# Autodesk Inventor assembly: UR5withBarrett
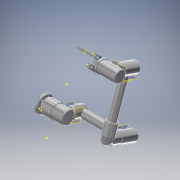
[picture p0: Inventor's stored thumbnail of the model, 180x180]
Saved by Autodesk Inventor 2016 (Build 200138000, 138)
## iProperties
Created: 2017-12-24
Part Number: UR5withBarrett
Document SubType Name: Assembly
Designer: kornbot
Author: kornbot
## Documents named in this file (15)
- C:\Users\kornbot\Documents\UR5withBarrett.iam
- C:\Users\kornbot\Documents\UR5 Joint base connection.ipt
- C:\Users\kornbot\Documents\UR5 base2.ipt
- C:\Users\kornbot\Documents\UR5 upper joint shoulder.ipt
- C:\Users\kornbot\Documents\UR5 joint shoulder 2.ipt
- C:\Users\kornbot\Documents\UR5 extended arm.ipt
- C:\Users\kornbot\Documents\UR5 joint elbow2.ipt
- C:\Users\kornbot\Documents\UR5 joint elbow3.ipt
- C:\Users\kornbot\Documents\UR5 Joint to wrist.ipt
- C:\Users\kornbot\Documents\UR5 End to wrist.ipt
- C:\Users\kornbot\Documents\UR5 Wrist Rotation.ipt
- C:\Users\kornbot\Documents\UR5 Palm.ipt
- C:\Users\kornbot\Documents\UR5 finger.ipt
- C:\Users\kornbot\Documents\UR5  finger lead.ipt
- C:\Users\kornbot\Documents\UR5 End finger.ipt
## Components (23 placed, 14 different names)
1. UR5 base2:1 — Rotational:1
2. UR5 Joint base connection:1 — Rotational:1, Rigid:1, Rigid:2
3. UR5 Joint base connection:2 — Rigid:1
4. UR5 upper joint shoulder:1 — Rigid:2, Rotational:2
5. UR5 joint shoulder 2:1 — Rotational:2, Rigid:3
6. UR5 joint shoulder 2:2 — Rigid:3, Rotational:3
7. UR5 extended arm:1 — Rotational:3, Rigid:4
8. UR5 joint elbow3:1 — Rigid:4, Rotational:4
9. UR5 Joint to wrist:1 — Rotational:4, Rigid:5
10. UR5 End to wrist:1 — Rigid:5, Rigid:6
11. UR5 joint elbow2:1 — Rigid:6, Rotational:5
12. UR5 joint elbow2:2 — Rotational:5, Rotational:6
13. UR5 Wrist Rotation:1 — Rotational:6, Rotational:7
14. UR5 Palm:1 — Rotational:7, Rotational:8, Rotational:9, Rigid:7
15. UR5 finger:1 — Rotational:9, Rotational:12
16. UR5 finger:2 — Rigid:7, Rotational:10
17. UR5 finger:3 — Rotational:8, Rotational:11
18. UR5  finger lead:1 — Rotational:10, Rotational:13
19. UR5  finger lead:2 — Rotational:12, Rotational:15
20. UR5  finger lead:3 — Rotational:11, Rotational:14
21. UR5 End finger:1 — Rotational:13
22. UR5 End finger:2 — Rotational:14
23. UR5 End finger:3 — Rotational:15
## Relationships (22: RevoluteJoint 15, WeldJoint 7)
- Rotational:1 [RevoluteJoint]: UR5 base2:1 ↔ UR5 Joint base connection:1
- Rigid:1 [WeldJoint]: UR5 Joint base connection:1 ↔ UR5 Joint base connection:2
- Rigid:2 [WeldJoint]: UR5 Joint base connection:1 ↔ UR5 upper joint shoulder:1
- Rotational:2 [RevoluteJoint]: UR5 upper joint shoulder:1 ↔ UR5 joint shoulder 2:1
- Rigid:3 [WeldJoint]: UR5 joint shoulder 2:1 ↔ UR5 joint shoulder 2:2
- Rotational:3 [RevoluteJoint] (-9.25 mm): UR5 joint shoulder 2:2 ↔ UR5 extended arm:1
- Rigid:4 [WeldJoint] (21.75 mm): UR5 extended arm:1 ↔ UR5 joint elbow3:1
- Rotational:4 [RevoluteJoint]: UR5 joint elbow3:1 ↔ UR5 Joint to wrist:1
- Rigid:5 [WeldJoint]: UR5 Joint to wrist:1 ↔ UR5 End to wrist:1
- Rigid:6 [WeldJoint]: UR5 End to wrist:1 ↔ UR5 joint elbow2:1
- Rotational:5 [RevoluteJoint]: UR5 joint elbow2:1 ↔ UR5 joint elbow2:2
- Rotational:6 [RevoluteJoint] (-2 mm): UR5 joint elbow2:2 ↔ UR5 Wrist Rotation:1
- Rotational:7 [RevoluteJoint]: UR5 Wrist Rotation:1 ↔ UR5 Palm:1
- Rotational:8 [RevoluteJoint] (8 mm): UR5 Palm:1 ↔ UR5 finger:3
- Rotational:9 [RevoluteJoint] (2.75 mm): UR5 Palm:1 ↔ UR5 finger:1
- Rigid:7 [WeldJoint] (8.75 mm): UR5 Palm:1 ↔ UR5 finger:2
- Rotational:10 [RevoluteJoint] (-8 mm): UR5 finger:2 ↔ UR5  finger lead:1
- Rotational:11 [RevoluteJoint]: UR5 finger:3 ↔ UR5  finger lead:3
- Rotational:12 [RevoluteJoint]: UR5 finger:1 ↔ UR5  finger lead:2
- Rotational:13 [RevoluteJoint]: UR5  finger lead:1 ↔ UR5 End finger:1
- Rotational:14 [RevoluteJoint]: UR5  finger lead:3 ↔ UR5 End finger:2
- Rotational:15 [RevoluteJoint]: UR5  finger lead:2 ↔ UR5 End finger:3
